# Autodesk Inventor assembly: gantry_frame
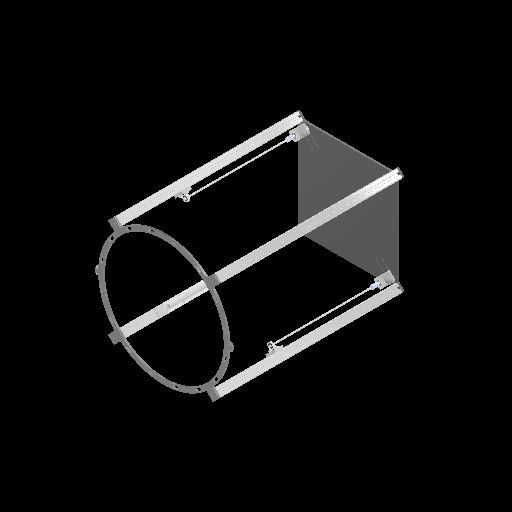
[picture p0: Inventor's stored thumbnail of the model, 512x512]
Saved by Autodesk Inventor 2026.1 (Build 301233000, 233)
## iProperties
Created: 2025-09-18
Part Number: gantry_frame
Document SubType Name: Assembly
Designer: drago
Author: drago
## Documents named in this file (6)
- C:\Users\drago\Desktop\_QIST4500_Multidisciplinary_Team_Project\Proteox MX magnet positioner CAD\gantry_frame\gantry_frame.iam
- C:\Users\drago\Desktop\_QIST4500_Multidisciplinary_Team_Project\Proteox MX magnet positioner CAD\gantry_frame\square_bar.ipt
- C:\Users\drago\Desktop\_QIST4500_Multidisciplinary_Team_Project\Proteox MX magnet positioner CAD\gantry_frame\base_plate.ipt
- C:\Users\drago\Desktop\_QIST4500_Multidisciplinary_Team_Project\Proteox MX magnet positioner CAD\z_rail\z_rail.iam
- C:\Users\drago\Desktop\_QIST4500_Multidisciplinary_Team_Project\Proteox MX magnet positioner CAD\gantry_frame\full_ring.iam
- C:\Users\drago\Desktop\_QIST4500_Multidisciplinary_Team_Project\Proteox MX magnet positioner CAD\z_translator\z_translator.iam
## Components (10 placed, 5 different names)
1. full_ring:1 [sub-assembly] — Mate:60, Mate:61, Mate:70, Mate:71
2. base_plate:1 — Mate:65, Angle:2, Mate:66, Mate:67, Mate:68, Mate:69, Mate:72, Mate:73, Mate:74, Mate:75, Mate:80
3. z_rail:1 [sub-assembly] — Mate:68, Mate:73, Mate:76
4. z_rail:2 [sub-assembly] — Mate:69, Mate:74, Mate:77
5. z_translator:1 [sub-assembly] — Mate:67, Mate:78, Mate:80
6. z_translator:2 [sub-assembly] — Mate:66, Mate:75, Mate:79
7. square_bar:1 — Mate:70, Mate:71, Angle:3, Mate:72, Mate:77
8. square_bar:2 — Mate:79
9. square_bar:3 — Mate:76
10. square_bar:4 — Mate:78
## Component patterns: (4 elements, first: square_bar:1)
## Relationships (20: Mate 18, Angle 2)
- Mate:60: full_ring:1
- Mate:61: full_ring:1
- Mate:65: base_plate:1
- Angle:2 (45 deg): base_plate:1
- Mate:66: base_plate:1 ↔ z_translator:2
- Mate:67: base_plate:1 ↔ z_translator:1
- Mate:68: base_plate:1 ↔ z_rail:1
- Mate:69: base_plate:1 ↔ z_rail:2
- Mate:70: full_ring:1 ↔ square_bar:1
- Mate:71: full_ring:1 ↔ square_bar:1
- Angle:3 (45 deg): square_bar:1
- Mate:72: base_plate:1 ↔ square_bar:1
- Mate:73: base_plate:1 ↔ z_rail:1
- Mate:74: base_plate:1 ↔ z_rail:2
- Mate:75: base_plate:1 ↔ z_translator:2
- Mate:76: z_rail:1 ↔ square_bar:3
- Mate:77: z_rail:2 ↔ square_bar:1
- Mate:78: z_translator:1 ↔ square_bar:4
- Mate:79: z_translator:2 ↔ square_bar:2
- Mate:80: base_plate:1 ↔ z_translator:1
